# Autodesk Inventor assembly: testRoboRescue_Chassis_Frame
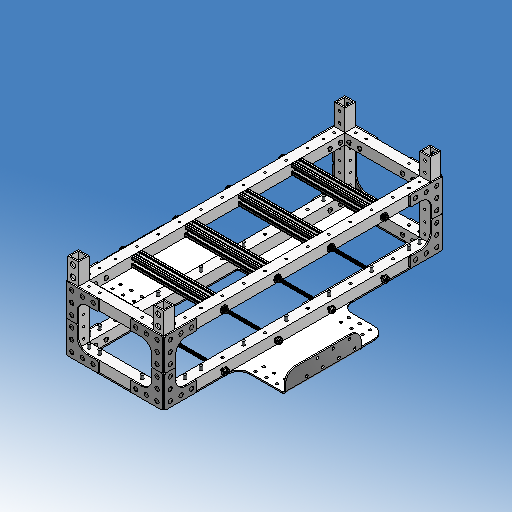
[picture p0: Inventor's stored thumbnail of the model, 512x512]
Saved by Autodesk Inventor 2025 (Build 290162000, 162)
## iProperties
Created: 2022-03-14
Part Number: testRoboRescue_Chassis_Frame
Document SubType Name: Assembly
Designer: Nebil Oumer
Mass: 5002.95 g
Surface Area: 15217.4 cm^2
Volume: 1975.13 cm^3
Density: 2.53297 g/cm^3
Author: Nebil Oumer
## Documents named in this file (17)
- C:\Users\seene\Desktop\Stony Brook\SBRT\RCR_Dexter\Chassis\Frame\Centerpiece\Centerpiece_Frame.iam
- Centerpiece_Frame.iam
- C:\Users\seene\Desktop\Stony Brook\SBRT\RCR_Dexter\Chassis\Frame\Centerpiece\Centerpiece_parts\Centerpiece_Frame_heightBar.ipt
- C:\Users\seene\Desktop\Stony Brook\SBRT\RCR_Dexter\Chassis\Frame\Centerpiece\Centerpiece_parts\Centerpiece_Frame_widthBar.ipt
- C:\Users\seene\Desktop\Stony Brook\SBRT\RCR_Dexter\Chassis\Frame\Centerpiece\Centerpiece_parts\Centerpiece_Frame_lengthBar.ipt
- C:\Users\seene\Desktop\Stony Brook\SBRT\RCR_Dexter\Chassis\Frame\Centerpiece\Centerpiece_parts\Centerpiece_bottomPlate.ipt
- C:\Users\seene\Desktop\Stony Brook\SBRT\RCR_Dexter\Chassis\Frame\Centerpiece\Centerpiece_parts\Centerpiece_FlatGusset.ipt
- C:\Users\seene\Desktop\Stony Brook\SBRT\RCR_Dexter\Chassis\Frame\Centerpiece\Centerpiece_parts\Rivet.ipt
- C:\Users\seene\Desktop\Stony Brook\SBRT\RCR_Dexter\Chassis\Frame\Centerpiece\Centerpiece_parts\Centerpiece_GussetBolt.ipt
- C:\Users\seene\Desktop\Stony Brook\SBRT\RCR_Dexter\Chassis\Frame\Centerpiece\Centerpiece_parts\Centerpiece_GussetBolt_MIR.ipt
- C:\Users\seene\Desktop\Stony Brook\SBRT\RCR_Dexter\Chassis\Frame\Centerpiece\Centerpiece_parts\Centerpiece_Frame_BottomLengthBar.ipt
- C:\Users\seene\Desktop\Stony Brook\SBRT\RCR_Dexter\Chassis\Frame\Centerpiece\Centerpiece_parts\Centerpiece_Frame_BottomWidthBar.ipt
- C:\Users\seene\Desktop\Stony Brook\SBRT\RCR_Dexter\Chassis\Frame\Centerpiece\Centerpiece_parts\T-Slotted Framing.ipt
- C:\Users\seene\Desktop\Stony Brook\SBRT\RCR_Dexter\Chassis\Chassis Frame\95412A316_18-8 Stainless Steel Threaded Rod.ipt
- C:\Users\seene\Desktop\Stony Brook\SBRT\RCR_Dexter\Chassis\Chassis Frame\91259A585_Alloy Steel Shoulder Screw.ipt
- C:\Users\seene\Desktop\Stony Brook\SBRT\RCR_Dexter\Chassis\Chassis Frame\96282A101_High-Strength Steel Serrated Flange Locknut.ipt
- C:\Users\seene\Desktop\Stony Brook\SBRT\RCR_Dexter\Chassis\Chassis Frame\rubberWasher1.ipt
## Components (195 placed, 15 different names)
1. Centerpiece_bottomPlate:1 — Mate:118, Mate:119, Mate:120, Mate:122, Mate:124, Mate:126, Mate:128, Mate:131, Mate:134, Mate:137, Mate:148
2. Centerpiece_Frame_heightBar:1 — Flush:36, Mate:18, Mate:25, Flush:51, Mate:26, Flush:52, Mate:27, Flush:55, Mate:28, Flush:74, Mate:43, Flush:75
3. Centerpiece_Frame_heightBar:2 — Flush:38, Flush:40, Flush:58, Mate:30, Flush:61, Mate:31, Flush:62, Mate:32, Flush:65, Mate:42, Mate:133
4. Centerpiece_Frame_heightBar:3 — Flush:31, Mate:21, Flush:42, Mate:22, Flush:44, Mate:23, Flush:46, Mate:24, Flush:48, Mate:41, Mate:127, Mate:136, Mate:139
5. Centerpiece_Frame_heightBar:4 — Mate:17, Flush:34, Mate:33, Flush:67, Mate:34, Mate:35, Flush:69, Mate:36, Flush:71, Mate:45, Flush:77, Mate:130
6. Centerpiece_Frame_BottomWidthBar:2 — Mate:136, Mate:137, Mate:138, Mate:145, Mate:146, Mate:147, Mate:159, Mate:161
7. Centerpiece_Frame_BottomWidthBar:1 — Mate:133, Mate:134, Mate:135, Mate:149, Mate:150, Mate:163
8. Centerpiece_Frame_widthBar:3 — Flush:8, Flush:40, Mate:29, Flush:59, Mate:43, Flush:75, Mate:157, Mate:165
9. Centerpiece_Frame_widthBar:4 — Flush:101, Mate:139, Flush:102, Mate:141, Mate:142, Mate:151, Mate:152
10. Centerpiece_Frame_BottomLengthBar:1 — Mate:127, Mate:128, Mate:129, Mate:143, Mate:144
11. Centerpiece_Frame_BottomLengthBar:2 — Mate:130, Mate:131, Mate:132
12. Centerpiece_Frame_lengthBar:1 — Mate:17, Flush:34, Flush:38, Flush:63, Flush:66, Mate:42, Symmetry:2, Flush:102
13. Centerpiece_Frame_lengthBar:4 — Flush:8, Flush:31, Flush:36, Mate:18, Flush:50, Flush:74, Mate:41, Flush:101
14. Centerpiece-FlatGusset:1 — Mate:25, Flush:50, Flush:51, Flush:53, Mate:108, Mate:109
15. Centerpiece-FlatGusset:2 — Mate:21, Flush:42, Flush:47, Mate:49, Mate:50, Mate:106, Mate:107
16. Centerpiece-FlatGusset:3 — Mate:23, Flush:46, Flush:47, Mate:51, Mate:52
17. Centerpiece-FlatGusset:4 — Mate:24, Flush:48, Flush:49, Mate:129
18. Centerpiece-FlatGusset:5 — Mate:29, Flush:58, Flush:59
19. Centerpiece-FlatGusset:6 — Mate:34, Flush:72, Mate:45, Flush:77, Mate:132
20. Centerpiece-FlatGusset:7 — Mate:28
21. Centerpiece-FlatGusset:8 — Mate:22, Flush:44, Flush:49, Mate:138
22. Centerpiece-FlatGusset:9 — Mate:27, Flush:55
23. Centerpiece-FlatGusset:10 — Mate:32, Flush:65
24. Centerpiece-FlatGusset:11 — Mate:36, Flush:71, Flush:72
25. Centerpiece-FlatGusset:12 — Mate:31, Flush:62, Flush:63, Mate:55, Mate:56, Mate:112, Mate:113
26. Centerpiece-FlatGusset:13 — Mate:26, Flush:52, Flush:53, Mate:53, Mate:54, Mate:110, Mate:111
27. Centerpiece-FlatGusset:14 — Mate:33, Flush:66, Flush:67, Flush:70
28. Centerpiece-FlatGusset:15 — Mate:30, Flush:61, Mate:135
29. Centerpiece-FlatGusset:16 — Mate:35, Flush:69, Flush:70
30. Centerpiece_GussetBolt_MIR:5 — Mate:146, Flush:103
31. Centerpiece_GussetBolt_MIR:6 — Mate:147, Mate:148, Flush:103, Flush:105
32. Centerpiece_GussetBolt_MIR:7 — Flush:104, Mate:149
33. Centerpiece_GussetBolt_MIR:8 — Flush:104, Flush:105, Mate:150
34. T-Slotted Framing:1 — Mate:141, Mate:142
35. T-Slotted Framing:2
36. T-Slotted Framing:3
37. T-Slotted Framing:4
38. 95412A316_18-8 Stainless Steel Threaded Rod:4 — Mate:159, Mate:160, Mate:162, Mate:164
39. 91259A585_Alloy Steel Shoulder Screw:3 — Mate:155, Mate:156, Mate:157
40. rubberWasher1:3 — Mate:155, Mate:156, Mate:165
41. rubberWasher1:4 — Mate:153, Mate:154
42. 91259A585_Alloy Steel Shoulder Screw:5 — Mate:151, Mate:152, Mate:153, Mate:154
43. 96282A101_High-Strength Steel Serrated Flange Locknut:5 — Mate:160, Mate:161, Mate:164
44. 96282A101_High-Strength Steel Serrated Flange Locknut:8 — Mate:162, Mate:163
45. 95412A316_18-8 Stainless Steel Threaded Rod:5
46. 91259A585_Alloy Steel Shoulder Screw:6
47. rubberWasher1:5
48. rubberWasher1:6
49. 91259A585_Alloy Steel Shoulder Screw:7
50. 96282A101_High-Strength Steel Serrated Flange Locknut:9
51. 96282A101_High-Strength Steel Serrated Flange Locknut:10
52. 95412A316_18-8 Stainless Steel Threaded Rod:6
53. 91259A585_Alloy Steel Shoulder Screw:8
54. rubberWasher1:7
55. rubberWasher1:8
56. 91259A585_Alloy Steel Shoulder Screw:9
57. 96282A101_High-Strength Steel Serrated Flange Locknut:11
58. 96282A101_High-Strength Steel Serrated Flange Locknut:12
59. 95412A316_18-8 Stainless Steel Threaded Rod:7
60. 91259A585_Alloy Steel Shoulder Screw:10
61. rubberWasher1:9
62. rubberWasher1:10
63. 91259A585_Alloy Steel Shoulder Screw:11
64. 96282A101_High-Strength Steel Serrated Flange Locknut:13
65. 96282A101_High-Strength Steel Serrated Flange Locknut:14
66. Centerpiece_GussetBolt:8 — Mate:124
67. Centerpiece_GussetBolt:7 — Mate:126
68. Centerpiece_GussetBolt:9 — Mate:143
69. Centerpiece_GussetBolt:10 — Mate:144
70. Centerpiece_GussetBolt:6 — Mate:122, Mate:145
71. Centerpiece_GussetBolt:5 — Mate:120
72. Centerpiece_GussetBolt:11
73. Centerpiece_GussetBolt:12
74. Centerpiece_GussetBolt:1 — Mate:118, Mate:119
75. Centerpiece_GussetBolt:13
76. Centerpiece_GussetBolt:14
77. Centerpiece_GussetBolt:15
78. Centerpiece_GussetBolt:16
79. Centerpiece_GussetBolt:17
80. Centerpiece_GussetBolt:18
81. Centerpiece_GussetBolt:19
82. Centerpiece_GussetBolt:20
83. Centerpiece_GussetBolt:21
84. Rivet:1 — Mate:49, Mate:50
85. Rivet:2
86. Rivet:3
87. Rivet:4
88. Rivet:5
89. Rivet:6
90. Rivet:13
91. Rivet:14
92. Rivet:15
93. Rivet:16
94. Rivet:17
95. Rivet:18
96. Rivet:7 — Mate:51, Mate:52
97. Rivet:8
98. Rivet:9
99. Rivet:10
100. Rivet:11
101. Rivet:12
102. Rivet:19
103. Rivet:20
104. Rivet:21
105. Rivet:22
106. Rivet:23
107. Rivet:24
108. Rivet:25 — Mate:53, Mate:54
109. Rivet:27
110. Rivet:28
111. Rivet:29
112. Rivet:30
113. Rivet:31
114. Rivet:32
115. Rivet:33
116. Rivet:34
117. Rivet:35
118. Rivet:36
119. Rivet:37
120. Rivet:26 — Mate:55, Mate:56
121. Rivet:38
122. Rivet:39
123. Rivet:40
124. Rivet:41
125. Rivet:42
126. Rivet:43
127. Rivet:44
128. Rivet:45
129. Rivet:46
130. Rivet:47
131. Rivet:48
132. Rivet:49 — Mate:106, Mate:107
133. Rivet:53
134. Rivet:54
135. Rivet:55
136. Rivet:56
137. Rivet:57
138. Rivet:58
139. Rivet:59
140. Rivet:81
141. Rivet:82
142. Rivet:83
143. Rivet:84
144. Rivet:85
145. Rivet:86
146. Rivet:87
147. Rivet:88
148. Rivet:51 — Mate:110, Mate:111
149. Rivet:74
150. Rivet:75
151. Rivet:76
152. Rivet:77
153. Rivet:78
154. Rivet:79
155. Rivet:80
156. Rivet:89
157. Rivet:90
158. Rivet:91
159. Rivet:92
160. Rivet:93
161. Rivet:94
162. Rivet:95
163. Rivet:96
164. Rivet:50 — Mate:108, Mate:109
165. Rivet:60
166. Rivet:61
167. Rivet:62
168. Rivet:63
169. Rivet:64
170. Rivet:65
171. Rivet:66
172. Rivet:97
173. Rivet:98
174. Rivet:99
175. Rivet:100
176. Rivet:101
177. Rivet:102
178. Rivet:103
179. Rivet:104
180. Rivet:52 — Mate:112, Mate:113
181. Rivet:67
182. Rivet:68
183. Rivet:69
184. Rivet:70
185. Rivet:71
186. Rivet:72
187. Rivet:73
188. Rivet:105
189. Rivet:106
190. Rivet:107
191. Rivet:108
192. Rivet:109
193. Rivet:110
194. Rivet:111
195. Rivet:112
## Component patterns: (4 elements, first: T-Slotted Framing:1), (4 elements, first: 95412A316_18-8 Stainless Steel Threaded Rod:4 + 91259A585_Alloy Steel Shoulder Screw:3 + rubberWasher1:3 + rubberWasher1:4 + 91259A585_Alloy Steel Shoulder Screw:5 + 96282A101_High-Strength Steel Serrated Flange Locknut:5 + 96282A101_High-Strength Steel Serrated Flange Locknut:8), (2 elements), (2 elements), (2 elements), (2 elements), (2 elements), (2 elements), (2 elements), (2 elements), (2 elements, first: Centerpiece_GussetBolt:8 + Centerpiece_GussetBolt:7), (2 elements, first: Centerpiece_GussetBolt:6 + Centerpiece_GussetBolt:5), (10 elements, first: Centerpiece_GussetBolt:1), (6 elements, first: Rivet:1), Component Pattern 1:2 (6 elements), (6 elements, first: Rivet:7), Component Pattern 2:2 (6 elements), (6 elements, first: Rivet:25), Component Pattern 5:2 (6 elements), (6 elements, first: Rivet:26), Component Pattern 7:2 (6 elements), (2 elements), Component Pattern 13:2 (2 elements), (2 elements), Component Pattern 19:2 (2 elements), (2 elements), Component Pattern 15:2 (2 elements), (2 elements), Component Pattern 17:2 (2 elements), (4 elements, first: Rivet:49), Component Pattern 12:2 (4 elements), Component Pattern 12:3 (4 elements), Component Pattern 12:4 (4 elements), (4 elements, first: Rivet:51), Component Pattern 18:2 (4 elements), Component Pattern 18:3 (4 elements), Component Pattern 18:4 (4 elements), (4 elements, first: Rivet:50), Component Pattern 14:2 (4 elements), Component Pattern 14:3 (4 elements), Component Pattern 14:4 (4 elements), (4 elements, first: Rivet:52), Component Pattern 16:2 (4 elements), Component Pattern 16:3 (4 elements), Component Pattern 16:4 (4 elements)
## Relationships (119: Mate 81, Flush 37, Symmetry 1)
- Flush:8: Centerpiece_Frame_widthBar:3 ↔ Centerpiece_Frame_lengthBar:4
- Flush:31: Centerpiece_Frame_heightBar:3 ↔ Centerpiece_Frame_lengthBar:4
- Mate:17: Centerpiece_Frame_heightBar:4 ↔ Centerpiece_Frame_lengthBar:1
- Flush:34: Centerpiece_Frame_heightBar:4 ↔ Centerpiece_Frame_lengthBar:1
- Flush:36: Centerpiece_Frame_heightBar:1 ↔ Centerpiece_Frame_lengthBar:4
- Mate:18: Centerpiece_Frame_heightBar:1 ↔ Centerpiece_Frame_lengthBar:4
- Flush:38: Centerpiece_Frame_heightBar:2 ↔ Centerpiece_Frame_lengthBar:1
- Flush:40: Centerpiece_Frame_heightBar:2 ↔ Centerpiece_Frame_widthBar:3
- Mate:21: Centerpiece_Frame_heightBar:3 ↔ Centerpiece-FlatGusset:2
- Flush:42: Centerpiece_Frame_heightBar:3 ↔ Centerpiece-FlatGusset:2
- Mate:22: Centerpiece_Frame_heightBar:3 ↔ Centerpiece-FlatGusset:8
- Flush:44: Centerpiece_Frame_heightBar:3 ↔ Centerpiece-FlatGusset:8
- Mate:23: Centerpiece_Frame_heightBar:3 ↔ Centerpiece-FlatGusset:3
- Flush:46: Centerpiece_Frame_heightBar:3 ↔ Centerpiece-FlatGusset:3
- Flush:47: Centerpiece-FlatGusset:2 ↔ Centerpiece-FlatGusset:3
- Mate:24: Centerpiece_Frame_heightBar:3 ↔ Centerpiece-FlatGusset:4
- Flush:48: Centerpiece_Frame_heightBar:3 ↔ Centerpiece-FlatGusset:4
- Flush:49: Centerpiece-FlatGusset:4 ↔ Centerpiece-FlatGusset:8
- Mate:25: Centerpiece_Frame_heightBar:1 ↔ Centerpiece-FlatGusset:1
- Flush:50: Centerpiece_Frame_lengthBar:4 ↔ Centerpiece-FlatGusset:1
- Flush:51: Centerpiece_Frame_heightBar:1 ↔ Centerpiece-FlatGusset:1
- Mate:26: Centerpiece_Frame_heightBar:1 ↔ Centerpiece-FlatGusset:13
- Flush:52: Centerpiece_Frame_heightBar:1 ↔ Centerpiece-FlatGusset:13
- Flush:53: Centerpiece-FlatGusset:1 ↔ Centerpiece-FlatGusset:13
- Mate:27: Centerpiece_Frame_heightBar:1 ↔ Centerpiece-FlatGusset:9
- Flush:55: Centerpiece_Frame_heightBar:1 ↔ Centerpiece-FlatGusset:9
- Mate:28: Centerpiece_Frame_heightBar:1 ↔ Centerpiece-FlatGusset:7
- Mate:29: Centerpiece_Frame_widthBar:3 ↔ Centerpiece-FlatGusset:5
- Flush:58: Centerpiece_Frame_heightBar:2 ↔ Centerpiece-FlatGusset:5
- Flush:59: Centerpiece_Frame_widthBar:3 ↔ Centerpiece-FlatGusset:5
- Mate:30: Centerpiece_Frame_heightBar:2 ↔ Centerpiece-FlatGusset:15
- Flush:61: Centerpiece_Frame_heightBar:2 ↔ Centerpiece-FlatGusset:15
- Mate:31: Centerpiece_Frame_heightBar:2 ↔ Centerpiece-FlatGusset:12
- Flush:62: Centerpiece_Frame_heightBar:2 ↔ Centerpiece-FlatGusset:12
- Flush:63: Centerpiece_Frame_lengthBar:1 ↔ Centerpiece-FlatGusset:12
- Mate:32: Centerpiece_Frame_heightBar:2 ↔ Centerpiece-FlatGusset:10
- Flush:65: Centerpiece_Frame_heightBar:2 ↔ Centerpiece-FlatGusset:10
- Mate:33: Centerpiece_Frame_heightBar:4 ↔ Centerpiece-FlatGusset:14
- Flush:66: Centerpiece_Frame_lengthBar:1 ↔ Centerpiece-FlatGusset:14
- Flush:67: Centerpiece_Frame_heightBar:4 ↔ Centerpiece-FlatGusset:14
- Mate:34: Centerpiece_Frame_heightBar:4 ↔ Centerpiece-FlatGusset:6
- Mate:35: Centerpiece_Frame_heightBar:4 ↔ Centerpiece-FlatGusset:16
- Flush:69: Centerpiece_Frame_heightBar:4 ↔ Centerpiece-FlatGusset:16
- Flush:70: Centerpiece-FlatGusset:14 ↔ Centerpiece-FlatGusset:16
- Mate:36: Centerpiece_Frame_heightBar:4 ↔ Centerpiece-FlatGusset:11
- Flush:71: Centerpiece_Frame_heightBar:4 ↔ Centerpiece-FlatGusset:11
- Flush:72: Centerpiece-FlatGusset:6 ↔ Centerpiece-FlatGusset:11
- Flush:74 (-50.8 mm): Centerpiece_Frame_heightBar:1 ↔ Centerpiece_Frame_lengthBar:4
- Mate:41: Centerpiece_Frame_heightBar:3 ↔ Centerpiece_Frame_lengthBar:4
- Mate:42: Centerpiece_Frame_heightBar:2 ↔ Centerpiece_Frame_lengthBar:1
- Mate:43: Centerpiece_Frame_heightBar:1 ↔ Centerpiece_Frame_widthBar:3
- Flush:75: Centerpiece_Frame_heightBar:1 ↔ Centerpiece_Frame_widthBar:3
- Mate:45: Centerpiece_Frame_heightBar:4 ↔ Centerpiece-FlatGusset:6
- Flush:77: Centerpiece_Frame_heightBar:4 ↔ Centerpiece-FlatGusset:6
- Mate:49: Centerpiece-FlatGusset:2 ↔ Rivet:1
- Mate:50: Centerpiece-FlatGusset:2 ↔ Rivet:1
- Mate:51: Centerpiece-FlatGusset:3 ↔ Rivet:7
- Mate:52: Centerpiece-FlatGusset:3 ↔ Rivet:7
- Mate:53: Centerpiece-FlatGusset:13 ↔ Rivet:25
- Mate:54: Centerpiece-FlatGusset:13 ↔ Rivet:25
- Mate:55: Centerpiece-FlatGusset:12 ↔ Rivet:26
- Mate:56: Centerpiece-FlatGusset:12 ↔ Rivet:26
- Mate:106: Centerpiece-FlatGusset:2 ↔ Rivet:49
- Mate:107: Centerpiece-FlatGusset:2 ↔ Rivet:49
- Mate:108: Centerpiece-FlatGusset:1 ↔ Rivet:50
- Mate:109: Centerpiece-FlatGusset:1 ↔ Rivet:50
- Mate:110: Centerpiece-FlatGusset:13 ↔ Rivet:51
- Mate:111: Centerpiece-FlatGusset:13 ↔ Rivet:51
- Mate:112: Centerpiece-FlatGusset:12 ↔ Rivet:52
- Mate:113: Centerpiece-FlatGusset:12 ↔ Rivet:52
- Mate:118: Centerpiece_bottomPlate:1 ↔ Centerpiece_GussetBolt:1
- Mate:119: Centerpiece_bottomPlate:1 ↔ Centerpiece_GussetBolt:1
- Mate:120: Centerpiece_bottomPlate:1 ↔ Centerpiece_GussetBolt:5
- Mate:122: Centerpiece_bottomPlate:1 ↔ Centerpiece_GussetBolt:6
- Mate:124: Centerpiece_bottomPlate:1 ↔ Centerpiece_GussetBolt:8
- Mate:126: Centerpiece_bottomPlate:1 ↔ Centerpiece_GussetBolt:7
- Symmetry:2: Centerpiece_Frame_lengthBar:1
- Mate:127: Centerpiece_Frame_heightBar:3 ↔ Centerpiece_Frame_BottomLengthBar:1
- Mate:128: Centerpiece_bottomPlate:1 ↔ Centerpiece_Frame_BottomLengthBar:1
- Mate:129: Centerpiece_Frame_BottomLengthBar:1 ↔ Centerpiece-FlatGusset:4
- Mate:130: Centerpiece_Frame_heightBar:4 ↔ Centerpiece_Frame_BottomLengthBar:2
- Mate:131: Centerpiece_bottomPlate:1 ↔ Centerpiece_Frame_BottomLengthBar:2
- Mate:132: Centerpiece_Frame_BottomLengthBar:2 ↔ Centerpiece-FlatGusset:6
- Mate:133: Centerpiece_Frame_heightBar:2 ↔ Centerpiece_Frame_BottomWidthBar:1
- Mate:134: Centerpiece_bottomPlate:1 ↔ Centerpiece_Frame_BottomWidthBar:1
- Mate:135: Centerpiece_Frame_BottomWidthBar:1 ↔ Centerpiece-FlatGusset:15
- Mate:136: Centerpiece_Frame_heightBar:3 ↔ Centerpiece_Frame_BottomWidthBar:2
- Mate:137: Centerpiece_bottomPlate:1 ↔ Centerpiece_Frame_BottomWidthBar:2
- Mate:138: Centerpiece_Frame_BottomWidthBar:2 ↔ Centerpiece-FlatGusset:8
- Flush:101: Centerpiece_Frame_widthBar:4 ↔ Centerpiece_Frame_lengthBar:4
- Mate:139: Centerpiece_Frame_heightBar:3 ↔ Centerpiece_Frame_widthBar:4
- Flush:102: Centerpiece_Frame_widthBar:4 ↔ Centerpiece_Frame_lengthBar:1
- Mate:141: Centerpiece_Frame_widthBar:4 ↔ T-Slotted Framing:1
- Mate:142: Centerpiece_Frame_widthBar:4 ↔ T-Slotted Framing:1
- Mate:143: Centerpiece_Frame_BottomLengthBar:1 ↔ Centerpiece_GussetBolt:9
- Mate:144: Centerpiece_Frame_BottomLengthBar:1 ↔ Centerpiece_GussetBolt:10
- Mate:145: Centerpiece_Frame_BottomWidthBar:2 ↔ Centerpiece_GussetBolt:6
- Mate:146: Centerpiece_Frame_BottomWidthBar:2 ↔ Centerpiece_GussetBolt_MIR:5
- Mate:147: Centerpiece_Frame_BottomWidthBar:2 ↔ Centerpiece_GussetBolt_MIR:6
- Mate:148: Centerpiece_bottomPlate:1 ↔ Centerpiece_GussetBolt_MIR:6
- Flush:103: Centerpiece_GussetBolt_MIR:5 ↔ Centerpiece_GussetBolt_MIR:6
- Flush:104: Centerpiece_GussetBolt_MIR:7 ↔ Centerpiece_GussetBolt_MIR:8
- Flush:105: Centerpiece_GussetBolt_MIR:6 ↔ Centerpiece_GussetBolt_MIR:8
- Mate:149: Centerpiece_Frame_BottomWidthBar:1 ↔ Centerpiece_GussetBolt_MIR:7
- Mate:150: Centerpiece_Frame_BottomWidthBar:1 ↔ Centerpiece_GussetBolt_MIR:8
- Mate:151: Centerpiece_Frame_widthBar:4 ↔ 91259A585_Alloy Steel Shoulder Screw:5
- Mate:152 (4.7752 mm): Centerpiece_Frame_widthBar:4 ↔ 91259A585_Alloy Steel Shoulder Screw:5
- Mate:153: rubberWasher1:4 ↔ 91259A585_Alloy Steel Shoulder Screw:5
- Mate:154: rubberWasher1:4 ↔ 91259A585_Alloy Steel Shoulder Screw:5
- Mate:155: 91259A585_Alloy Steel Shoulder Screw:3 ↔ rubberWasher1:3
- Mate:156: 91259A585_Alloy Steel Shoulder Screw:3 ↔ rubberWasher1:3
- Mate:157: Centerpiece_Frame_widthBar:3 ↔ 91259A585_Alloy Steel Shoulder Screw:3
- Mate:159: Centerpiece_Frame_BottomWidthBar:2 ↔ 95412A316_18-8 Stainless Steel Threaded Rod:4
- Mate:160: 95412A316_18-8 Stainless Steel Threaded Rod:4 ↔ 96282A101_High-Strength Steel Serrated Flange Locknut:5
- Mate:161 (6.35 mm): Centerpiece_Frame_BottomWidthBar:2 ↔ 96282A101_High-Strength Steel Serrated Flange Locknut:5
- Mate:162: 95412A316_18-8 Stainless Steel Threaded Rod:4 ↔ 96282A101_High-Strength Steel Serrated Flange Locknut:8
- Mate:163 (6.35 mm): Centerpiece_Frame_BottomWidthBar:1 ↔ 96282A101_High-Strength Steel Serrated Flange Locknut:8
- Mate:164: 95412A316_18-8 Stainless Steel Threaded Rod:4 ↔ 96282A101_High-Strength Steel Serrated Flange Locknut:5
- Mate:165 (6.35 mm): Centerpiece_Frame_widthBar:3 ↔ rubberWasher1:3
